# Autodesk Inventor assembly: Siłowiec
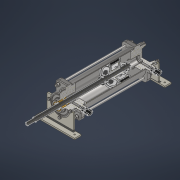
[picture p0: Inventor's stored thumbnail of the model, 180x180]
Saved by Autodesk Inventor 2022 (Build 260153000, 153)
## iProperties
Created: 2023-04-12
Part Number: Siłowiec
Document SubType Name: Assembly
Designer: jacek
Author: jacek
## Documents named in this file (18)
- D:\Pulpit\Silownik\Actuator\Siłowiec.iam
- D:\Pulpit\Silownik\Actuator\Łapa.iam
- D:\Pulpit\Silownik\Actuator\Pokrywa cylindra tyl.ipt
- D:\Pulpit\Silownik\Actuator\Uszczelka pokrywy.ipt
- D:\Pulpit\Silownik\Actuator\Cylinder.ipt
- D:\Pulpit\Silownik\Actuator\Pokrywa cylindra.ipt
- D:\Pulpit\Silownik\Actuator\tłoczysko.ipt
- D:\Pulpit\Silownik\Actuator\Tłok.ipt
- D:\Pulpit\Silownik\Actuator\Uszczelka.ipt
- D:\Pulpit\Silownik\Actuator\Pret mocujacy.ipt
- D:\Dokumenty\Inventor\Content Center Files\R2022\pl-PL\AS 1110\AS 1110 - M6 x 20.ipt
- D:\Dokumenty\Inventor\Content Center Files\R2022\pl-PL\AS 1968\AS 1968 - 1976 - 6.ipt
- D:\Dokumenty\Inventor\Content Center Files\R2022\pl-PL\AS 1968\AS 1968 - 1976 - 8.ipt
- D:\Dokumenty\Inventor\Content Center Files\R2022\pl-PL\AS 1112 (2)\AS 1112 - M8  Typ 10.ipt
- D:\Dokumenty\Inventor\Content Center Files\R2022\pl-PL\Parker A(28)\Parker A-Lok, gwint męski stożkowy - rura metryczna M14 x 1_4.ipt
- D:\Pulpit\Silownik\Actuator\Mocowanie uszczelki przod.ipt
- D:\Pulpit\Silownik\Actuator\Mocowanie uszczelki tyl.ipt
- D:\Pulpit\Silownik\Actuator\Uszczelka front.ipt
## Components (48 placed, 17 different names)
1. Łapa:1 [sub-assembly] — Zestawiające:1, Zestawiające:2, Zestawiające:3, Zestawiające:9, Wstawiające:6, Wstawiające:7, Wstawiające:8
2. Łapa:2 [sub-assembly] — Wstawiające:5, Wstawiające:9, Wstawiające:10, Wstawiające:11
3. AS 1110 - Metryczny M6 x 20:1 — Wstawiające:12
4. AS 1110 - Metryczny M6 x 20:2 — Wstawiające:13
5. AS 1110 - Metryczny M6 x 20:3 — Wstawiające:14
6. AS 1110 - Metryczny M6 x 20:4 — Wstawiające:15
7. AS 1110 - Metryczny M6 x 20:5 — Wstawiające:16
8. AS 1110 - Metryczny M6 x 20:6 — Wstawiające:17
9. AS 1968 6:1 — Wstawiające:6, Wstawiające:12
10. AS 1968 6:2 — Wstawiające:7, Wstawiające:13
11. AS 1968 6:3 — Wstawiające:8, Wstawiające:14
12. AS 1968 6:4 — Wstawiające:9, Wstawiające:16
13. AS 1968 6:5 — Wstawiające:10, Wstawiające:17
14. AS 1968 6:6 — Wstawiające:11, Wstawiające:15
15. Mocowanie uszczelki przod:1 — Wstawiające:34, Wstawiające:35, Sztywne:6
16. Mocowanie uszczelki tyl:1 — Wstawiające:36
17. Uszczelka front:1 — Wstawiające:35, Wstawiające:36
18. Uszczelka front:2 — Sztywne:6
19. Uszczelka pokrywy:1 — Wstawiające:1
20. Uszczelka pokrywy:2 — Wstawiające:3
21. Pokrywa cylindra tyl:1 — Zestawiające:1, Zestawiające:2, Zestawiające:3, Wstawiające:1, Wstawiające:2, Zestawiające:5, Zestawiające:6, Zestawiające:7, Zestawiające:8, Wstawiające:18, Wstawiające:19, Wstawiające:20, Wstawiające:21, Sztywne:3
22. Pokrywa cylindra:1 — Wstawiające:3, Wstawiające:4, Wstawiające:5, Wstawiające:22, Wstawiające:23, Wstawiające:24, Wstawiające:25, Sztywne:4, Wstawiające:34
23. Cylinder:1 — Wstawiające:2, Wstawiające:4, Zestawiające:4
24. Pret mocujacy:1 — Zestawiające:5, Równoległe:3
25. Pret mocujacy:2 — Zestawiające:6, Równoległe:1, Zestawiające:9
26. Pret mocujacy:3 — Zestawiające:7, Równoległe:1, Równoległe:2
27. Pret mocujacy:4 — Zestawiające:8, Równoległe:2, Równoległe:3
28. AS 1112 (2) - Metryczny M8  Typ 10:1 — Wstawiające:26
29. AS 1112 (2) - Metryczny M8  Typ 10:2 — Wstawiające:27
30. AS 1112 (2) - Metryczny M8  Typ 10:3 — Wstawiające:28
31. AS 1112 (2) - Metryczny M8  Typ 10:4 — Wstawiające:29
32. AS 1112 (2) - Metryczny M8  Typ 10:5 — Wstawiające:30
33. AS 1112 (2) - Metryczny M8  Typ 10:6 — Wstawiające:31
34. AS 1112 (2) - Metryczny M8  Typ 10:7 — Wstawiające:32
35. AS 1112 (2) - Metryczny M8  Typ 10:8 — Wstawiające:33
36. AS 1968 8:1 — Wstawiające:18, Wstawiające:30
37. AS 1968 8:2 — Wstawiające:19, Wstawiające:33
38. AS 1968 8:3 — Wstawiające:20, Wstawiające:32
39. AS 1968 8:4 — Wstawiające:21, Wstawiające:31
40. AS 1968 8:5 — Wstawiające:22, Wstawiające:26
41. AS 1968 8:6 — Wstawiające:23, Wstawiające:29
42. AS 1968 8:7 — Wstawiające:24, Wstawiające:27
43. AS 1968 8:8 — Wstawiające:25, Wstawiające:28
44. Tłok:1 — Sztywne:1, Sztywne:5
45. tłoczysko:1 — Sztywne:1
46. Uszczelka:1 — Zestawiające:4, Sztywne:5
47. Parker A-Lok, gwint męski stożkowy - rura metryczna M14 x 1/4:1 — Sztywne:3
48. Parker A-Lok, gwint męski stożkowy - rura metryczna M14 x 1/4:2 — Sztywne:4
## Relationships (53: Insert 36, Mate 9, WeldJoint 5, Flush 3)
- Zestawiające:1 [Mate]: Łapa:1 ↔ Pokrywa cylindra tyl:1
- Zestawiające:2 [Mate]: Łapa:1 ↔ Pokrywa cylindra tyl:1
- Zestawiające:3 [Mate]: Łapa:1 ↔ Pokrywa cylindra tyl:1
- Wstawiające:1 [Insert]: Uszczelka pokrywy:1 ↔ Pokrywa cylindra tyl:1
- Wstawiające:2 [Insert]: Pokrywa cylindra tyl:1 ↔ Cylinder:1
- Wstawiające:3 [Insert]: Uszczelka pokrywy:2 ↔ Pokrywa cylindra:1
- Wstawiające:4 [Insert]: Pokrywa cylindra:1 ↔ Cylinder:1
- Sztywne:1 [WeldJoint]: Tłok:1 ↔ tłoczysko:1
- Zestawiające:4 [Mate]: Cylinder:1 ↔ Uszczelka:1
- Zestawiające:5 [Mate]: Pokrywa cylindra tyl:1 ↔ Pret mocujacy:1
- Zestawiające:6 [Mate]: Pokrywa cylindra tyl:1 ↔ Pret mocujacy:2
- Zestawiające:7 [Mate]: Pokrywa cylindra tyl:1 ↔ Pret mocujacy:3
- Zestawiające:8 [Mate]: Pokrywa cylindra tyl:1 ↔ Pret mocujacy:4
- Równoległe:1 [Flush]: Pret mocujacy:2 ↔ Pret mocujacy:3
- Równoległe:2 [Flush]: Pret mocujacy:3 ↔ Pret mocujacy:4
- Równoległe:3 [Flush]: Pret mocujacy:1 ↔ Pret mocujacy:4
- Zestawiające:9 [Mate] (15 mm): Łapa:1 ↔ Pret mocujacy:2
- Wstawiające:5 [Insert]: Łapa:2 ↔ Pokrywa cylindra:1
- Wstawiające:6 [Insert]: Łapa:1 ↔ AS 1968 6:1
- Wstawiające:7 [Insert]: Łapa:1 ↔ AS 1968 6:2
- Wstawiające:8 [Insert]: Łapa:1 ↔ AS 1968 6:3
- Wstawiające:9 [Insert]: Łapa:2 ↔ AS 1968 6:4
- Wstawiające:10 [Insert]: Łapa:2 ↔ AS 1968 6:5
- Wstawiające:11 [Insert]: Łapa:2 ↔ AS 1968 6:6
- Wstawiające:12 [Insert]: AS 1110 - Metryczny M6 x 20:1 ↔ AS 1968 6:1
- Wstawiające:13 [Insert]: AS 1110 - Metryczny M6 x 20:2 ↔ AS 1968 6:2
- Wstawiające:14 [Insert]: AS 1110 - Metryczny M6 x 20:3 ↔ AS 1968 6:3
- Wstawiające:15 [Insert]: AS 1110 - Metryczny M6 x 20:4 ↔ AS 1968 6:6
- Wstawiające:16 [Insert]: AS 1110 - Metryczny M6 x 20:5 ↔ AS 1968 6:4
- Wstawiające:17 [Insert]: AS 1110 - Metryczny M6 x 20:6 ↔ AS 1968 6:5
- Wstawiające:18 [Insert]: Pokrywa cylindra tyl:1 ↔ AS 1968 8:1
- Wstawiające:19 [Insert]: Pokrywa cylindra tyl:1 ↔ AS 1968 8:2
- Wstawiające:20 [Insert]: Pokrywa cylindra tyl:1 ↔ AS 1968 8:3
- Wstawiające:21 [Insert]: Pokrywa cylindra tyl:1 ↔ AS 1968 8:4
- Wstawiające:22 [Insert]: Pokrywa cylindra:1 ↔ AS 1968 8:5
- Wstawiające:23 [Insert]: Pokrywa cylindra:1 ↔ AS 1968 8:6
- Wstawiające:24 [Insert]: Pokrywa cylindra:1 ↔ AS 1968 8:7
- Wstawiające:25 [Insert]: Pokrywa cylindra:1 ↔ AS 1968 8:8
- Wstawiające:26 [Insert]: AS 1112 (2) - Metryczny M8  Typ 10:1 ↔ AS 1968 8:5
- Wstawiające:27 [Insert]: AS 1112 (2) - Metryczny M8  Typ 10:2 ↔ AS 1968 8:7
- Wstawiające:28 [Insert]: AS 1112 (2) - Metryczny M8  Typ 10:3 ↔ AS 1968 8:8
- Wstawiające:29 [Insert]: AS 1112 (2) - Metryczny M8  Typ 10:4 ↔ AS 1968 8:6
- Wstawiające:30 [Insert]: AS 1112 (2) - Metryczny M8  Typ 10:5 ↔ AS 1968 8:1
- Wstawiające:31 [Insert]: AS 1112 (2) - Metryczny M8  Typ 10:6 ↔ AS 1968 8:4
- Wstawiające:32 [Insert]: AS 1112 (2) - Metryczny M8  Typ 10:7 ↔ AS 1968 8:3
- Wstawiające:33 [Insert]: AS 1112 (2) - Metryczny M8  Typ 10:8 ↔ AS 1968 8:2
- Sztywne:3 [WeldJoint]: Pokrywa cylindra tyl:1 ↔ Parker A-Lok, gwint męski stożkowy - rura metryczna M14 x 1/4:1
- Sztywne:4 [WeldJoint]: Pokrywa cylindra:1 ↔ Parker A-Lok, gwint męski stożkowy - rura metryczna M14 x 1/4:2
- Sztywne:5 [WeldJoint]: Tłok:1 ↔ Uszczelka:1
- Wstawiające:34 [Insert]: Mocowanie uszczelki przod:1 ↔ Pokrywa cylindra:1
- Wstawiające:35 [Insert]: Mocowanie uszczelki przod:1 ↔ Uszczelka front:1
- Wstawiające:36 [Insert]: Mocowanie uszczelki tyl:1 ↔ Uszczelka front:1
- Sztywne:6 [WeldJoint]: Mocowanie uszczelki przod:1 ↔ Uszczelka front:2
